# Autodesk Inventor assembly: SENSOR BRACKET RevC
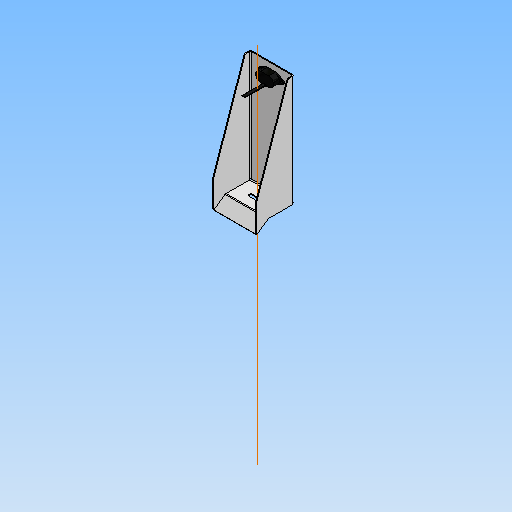
[picture p0: Inventor's stored thumbnail of the model, 512x512]
Saved by Autodesk Inventor 2025.3 (Build 293356000, 356)
## iProperties
Created: 2025-10-16
Part Number: SENSOR BRACKET RevC
Document SubType Name: Assembly
Designer: josh
Mass: 255.011 g
Surface Area: 816.272 cm^2
Volume: 71.9666 cm^3
Density: 3.54346 g/cm^3
Author: josh
## Documents named in this file (3)
- C:\WORK\INVENTOR PROJECTS\misc custom projects\O&M ROBOTICS\SENSOR BRACKET RevC.iam
- C:\WORK\INVENTOR PROJECTS\misc custom projects\O&M ROBOTICS\OM_CAGE-017.ipt
- C:\WORK\INVENTOR PROJECTS\misc custom projects\O&M ROBOTICS\Cage Sensor.ipt
## Components (2 placed, 2 different names)
1. OM_CAGE-017:1 — Insert:1, Insert:2
2. Cage Sensor:1 — Insert:1, Insert:2
## Relationships (2: Insert 2)
- Insert:1: OM_CAGE-017:1 ↔ Cage Sensor:1
- Insert:2: OM_CAGE-017:1 ↔ Cage Sensor:1
